# Autodesk Inventor assembly: forma
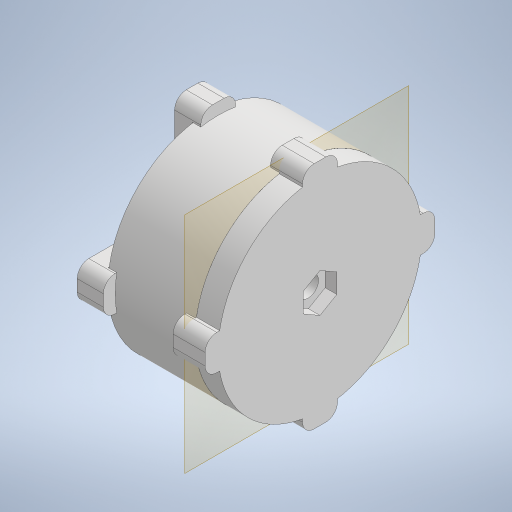
[picture p0: Inventor's stored thumbnail of the model, 512x512]
Saved by Autodesk Inventor 2023 (Build 270158000, 158)
## iProperties
Created: 2023-08-20
Part Number: forma
Document SubType Name: Assembly
Designer: Kamil
Author: Kamil
## Documents named in this file (6)
- C:\Users\Kamil\Desktop\MojeRoboty\Stefan\mechanics 2\forma.iam
- C:\Users\Kamil\Desktop\MojeRoboty\Stefan\mechanics 2\opona.ipt
- C:\Users\Kamil\Desktop\kolo.ipt
- C:\Users\Kamil\Desktop\MojeRoboty\Stefan\mechanics 2\podstawa_formy.ipt
- C:\Users\Kamil\Desktop\MojeRoboty\Stefan\mechanics 2\gora.ipt
- C:\Users\Kamil\Desktop\MojeRoboty\Stefan\mechanics 2\dol.ipt
## Components (5 placed, 5 different names)
1. opona:1 — Równoległe:1, Zestawiające:1, Równoległe:2
2. kolo:1 — Równoległe:1, Zestawiające:1
3. podstawa_formy:1 — Równoległe:2, Równoległe:3, Równoległe:4, Równoległe:5
4. gora:1 — Równoległe:3
5. dol:1 — Równoległe:4, Równoległe:5
## Relationships (6: Flush 5, Mate 1)
- Równoległe:1 [Flush]: opona:1 ↔ kolo:1
- Zestawiające:1 [Mate]: opona:1 ↔ kolo:1
- Równoległe:2 [Flush]: opona:1 ↔ podstawa_formy:1
- Równoległe:3 [Flush]: podstawa_formy:1 ↔ gora:1
- Równoległe:4 [Flush]: podstawa_formy:1 ↔ dol:1
- Równoległe:5 [Flush]: podstawa_formy:1 ↔ dol:1
